# Autodesk Inventor assembly: Pneumatics Mounted in Undercarriage
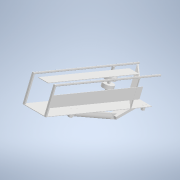
[picture p0: Inventor's stored thumbnail of the model, 180x180]
Saved by Autodesk Inventor 2020 (Build 240168000, 168)
## iProperties
Created: 2021-01-30
Part Number: Pneumatics Mounted in Undercarriage
Document SubType Name: Assembly
Designer: magda
Author: magda
## Documents named in this file (11)
- C:\Users\magda\OneDrive\Documents\Inventor\T3\Ramp Intake\Pneumatics Mounted in Undercarriage.iam
- C:\Users\magda\OneDrive\Documents\Inventor\T3\Ramp Intake\Undercarriage load and pannel.iam
- C:\Users\magda\OneDrive\Documents\Inventor\T3\Ramp Intake\Pneumatics Assembly.iam
- C:\Users\magda\OneDrive\Documents\Inventor\T3\Ramp Intake\Main Axle notch.ipt
- C:\Users\magda\OneDrive\Documents\Inventor\T3\Ramp Intake\Main Axle.ipt
- C:\Users\magda\OneDrive\Documents\Inventor\T3\Ramp Intake\Ramp Base.ipt
- C:\Users\magda\OneDrive\Documents\Inventor\T3\Ramp Intake\PVC Line.ipt
- C:\Users\magda\OneDrive\Documents\Inventor\T3\Ramp Intake\Part Joint.ipt
- C:\Users\magda\OneDrive\Documents\Inventor\T3\Ramp Intake\Redirection Plate.ipt
- C:\Users\magda\OneDrive\Documents\Inventor\T3\Ramp Intake\Random Compliance Wheel.ipt
- C:\Users\magda\OneDrive\Documents\Inventor\T3\Ramp Intake\Side Shield.ipt
## Components (16 placed, 10 different names)
1. Undercarriage load and pannel:1 [sub-assembly] — Mate:1, Mate:2, Mate:3, Mate:4, Mate:5, Mate:6, Mate:7, Mate:8, Flush:2, Flush:3, Flush:4, Flush:5, Mate:14, Flush:6, Flush:7, Mate:15, Flush:8, Flush:9, Mate:18, Flush:11, Flush:12, Mate:19, Flush:13, Flush:14, Mate:24, Mate:25, Flush:15, Mate:26, Mate:27, Flush:18
2. Pneumatics Assembly:1 [sub-assembly] — Mate:1, Mate:2, Mate:11, Mate:12
3. Main Axle notch:1 — Mate:3, Mate:4, Mate:5
4. Main Axle notch:2 — Mate:6, Mate:7, Mate:8, Flush:1, Mate:9
5. Main Axle:1 — Flush:1, Mate:9, Mate:13
6. Ramp Base:1 — Mate:11, Mate:12, Mate:13
7. PVC Line:1 — Flush:2, Flush:4, Mate:16, Flush:10
8. PVC Line:2 — Flush:3, Flush:5, Mate:17, Flush:17
9. Part Joint:1 — Mate:14, Flush:6, Flush:7, Mate:17, Flush:16
10. Part Joint:2 — Mate:15, Flush:8, Flush:9, Mate:16, Flush:10
11. Redirection Plate:1 — Mate:18, Flush:11, Flush:12
12. Part Joint:3 — Mate:19, Flush:13, Flush:14, Mate:20, Mate:21, Mate:22, Mate:23
13. Random Compliance Wheel:1 — Mate:20, Mate:21, Mate:24
14. Random Compliance Wheel:2 — Mate:22, Mate:23, Mate:25
15. Side Shield:1 — Flush:15, Mate:26, Flush:16
16. Side Shield:2 — Mate:27, Flush:17, Flush:18
## Relationships (44: Mate 26, Flush 18)
- Mate:1: Undercarriage load and pannel:1 ↔ Pneumatics Assembly:1
- Mate:2: Undercarriage load and pannel:1 ↔ Pneumatics Assembly:1
- Mate:3: Undercarriage load and pannel:1 ↔ Main Axle notch:1
- Mate:4: Undercarriage load and pannel:1 ↔ Main Axle notch:1
- Mate:5: Undercarriage load and pannel:1 ↔ Main Axle notch:1
- Mate:6: Undercarriage load and pannel:1 ↔ Main Axle notch:2
- Mate:7: Undercarriage load and pannel:1 ↔ Main Axle notch:2
- Mate:8: Undercarriage load and pannel:1 ↔ Main Axle notch:2
- Flush:1: Main Axle notch:2 ↔ Main Axle:1
- Mate:9: Main Axle notch:2 ↔ Main Axle:1
- Mate:11: Pneumatics Assembly:1 ↔ Ramp Base:1
- Mate:12: Pneumatics Assembly:1 ↔ Ramp Base:1
- Mate:13: Main Axle:1 ↔ Ramp Base:1
- Flush:2: Undercarriage load and pannel:1 ↔ PVC Line:1
- Flush:3: Undercarriage load and pannel:1 ↔ PVC Line:2
- Flush:4: Undercarriage load and pannel:1 ↔ PVC Line:1
- Flush:5: Undercarriage load and pannel:1 ↔ PVC Line:2
- Mate:14: Undercarriage load and pannel:1 ↔ Part Joint:1
- Flush:6: Undercarriage load and pannel:1 ↔ Part Joint:1
- Flush:7: Undercarriage load and pannel:1 ↔ Part Joint:1
- Mate:15: Undercarriage load and pannel:1 ↔ Part Joint:2
- Flush:8: Undercarriage load and pannel:1 ↔ Part Joint:2
- Flush:9: Undercarriage load and pannel:1 ↔ Part Joint:2
- Mate:16: PVC Line:1 ↔ Part Joint:2
- Flush:10: PVC Line:1 ↔ Part Joint:2
- Mate:17: PVC Line:2 ↔ Part Joint:1
- Mate:18: Undercarriage load and pannel:1 ↔ Redirection Plate:1
- Flush:11: Undercarriage load and pannel:1 ↔ Redirection Plate:1
- Flush:12: Undercarriage load and pannel:1 ↔ Redirection Plate:1
- Mate:19: Undercarriage load and pannel:1 ↔ Part Joint:3
- Flush:13: Undercarriage load and pannel:1 ↔ Part Joint:3
- Flush:14 (203.2 mm): Undercarriage load and pannel:1 ↔ Part Joint:3
- Mate:20: Part Joint:3 ↔ Random Compliance Wheel:1
- Mate:21: Part Joint:3 ↔ Random Compliance Wheel:1
- Mate:22: Part Joint:3 ↔ Random Compliance Wheel:2
- Mate:23: Part Joint:3 ↔ Random Compliance Wheel:2
- Mate:24 (50.8 mm): Undercarriage load and pannel:1 ↔ Random Compliance Wheel:1
- Mate:25 (101.6 mm): Undercarriage load and pannel:1 ↔ Random Compliance Wheel:2
- Flush:15: Undercarriage load and pannel:1 ↔ Side Shield:1
- Mate:26 (50.8 mm): Undercarriage load and pannel:1 ↔ Side Shield:1
- Flush:16: Part Joint:1 ↔ Side Shield:1
- Mate:27 (177.8 mm): Undercarriage load and pannel:1 ↔ Side Shield:2
- Flush:17 (50.8 mm): PVC Line:2 ↔ Side Shield:2
- Flush:18: Undercarriage load and pannel:1 ↔ Side Shield:2
